# Autodesk Inventor assembly: Ball Shifter Shafty assy
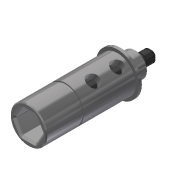
[picture p0: Inventor's stored thumbnail of the model, 180x180]
Saved by Autodesk Inventor 2013 (Build 170138000, 138)
## iProperties
Created: 2013-04-08
Part Number: Ball Shifter Shafty assy
Document SubType Name: Assembly
Designer: Niemitalo_Dan
Author: Niemitalo_Dan
## Documents named in this file (3)
- H:\Nemo\Documents\Robotics\COTS Parts\Gearboxes\Components\Ballshifter\Ball Shifter Shaft assy.iam
- H:\Nemo\Documents\Robotics\COTS Parts\Gearboxes\Components\Ballshifter\BallShifter ball housing.ipt
- H:\Nemo\Documents\Robotics\COTS Parts\Gearboxes\Components\Ballshifter\Ball shifting shaft.ipt
## Components (2 placed, 2 different names)
1. BallShifter ball housing:1 — Mate:1, Flush:1
2. Ball shifting shaft:1 — Mate:1, Flush:1
## Relationships (2: Mate 1, Flush 1)
- Mate:1: BallShifter ball housing:1 ↔ Ball shifting shaft:1
- Flush:1 (8.382 mm): BallShifter ball housing:1 ↔ Ball shifting shaft:1
